# Autodesk Inventor assembly: McCrea_kos_walle
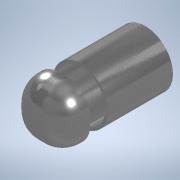
[picture p0: Inventor's stored thumbnail of the model, 180x180]
Saved by Autodesk Inventor 2022 (Build 260153000, 153)
## iProperties
Created: 2022-02-09
Part Number: McCrea_kos_walle
Document SubType Name: Assembly
Designer: Max
Author: Max
## Documents named in this file (5)
- C:\Users\Max\Documents\Inventor\Mold Design1\McCrea_kos_walle.iam
- C:\Users\Max\Documents\Inventor\Mold Design1\McCrea_kos_walle_McCrea_horny_kos_walle_LY.iam
- C:\Users\Max\Documents\Inventor\Mold Design1\McCrea_kos_walle_McCrea_obdlznicky_kos_walle_LY.iam
- C:\Users\Max\Documents\Škola\teg\Wall-e\maxo\McCrea_dolny_kos_walle.ipt
- C:\Users\Max\Documents\Škola\teg\Wall-e\maxo\McCrea_obdlznicky_kos_walle.ipt
## Components (6 placed, 4 different names)
1. McCrea_kos_walle_McCrea_horny_kos_walle_LY:1 [sub-assembly] — Rigid:1, Rigid:2, Rigid:3, Rigid:4
2. McCrea_kos_walle_McCrea_obdlznicky_kos_walle_LY:1 [sub-assembly] — Rigid:2
3. McCrea_kos_walle_McCrea_obdlznicky_kos_walle_LY:3 [sub-assembly] — Rigid:4, Mate:1
4. McCrea_kos_walle_McCrea_obdlznicky_kos_walle_LY:4 [sub-assembly] — Rigid:3
5. McCrea_obdlznicky_kos_walle:1 — Rigid:1
6. McCrea_dolny_kos_walle:1 — Mate:1
## Relationships (5: WeldJoint 4, Mate 1)
- Rigid:1 [WeldJoint]: McCrea_kos_walle_McCrea_horny_kos_walle_LY:1 ↔ McCrea_obdlznicky_kos_walle:1
- Rigid:2 [WeldJoint]: McCrea_kos_walle_McCrea_horny_kos_walle_LY:1 ↔ McCrea_kos_walle_McCrea_obdlznicky_kos_walle_LY:1
- Rigid:3 [WeldJoint]: McCrea_kos_walle_McCrea_horny_kos_walle_LY:1 ↔ McCrea_kos_walle_McCrea_obdlznicky_kos_walle_LY:4
- Rigid:4 [WeldJoint]: McCrea_kos_walle_McCrea_horny_kos_walle_LY:1 ↔ McCrea_kos_walle_McCrea_obdlznicky_kos_walle_LY:3
- Mate:1: McCrea_kos_walle_McCrea_obdlznicky_kos_walle_LY:3 ↔ McCrea_dolny_kos_walle:1
